# Autodesk Inventor assembly: Motor-Assembly
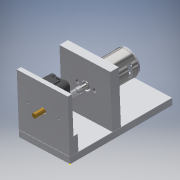
[picture p0: Inventor's stored thumbnail of the model, 180x180]
Saved by Autodesk Inventor 2016 (Build 200138000, 138)
## iProperties
Created: 2015-05-19
Part Number: Motor-Assembly
Document SubType Name: Assembly
Designer: jonathan
Author: jonathan
## Documents named in this file (3)
- C:\Users\jonathan\Desktop\CLEAN COPIES\DC Motor Test Stand\Inventor\DC Motor Test Stand.iam
- C:\Users\jonathan\Desktop\CLEAN COPIES\DC Motor Test Stand\Inventor\Fixture Assembly.iam
- C:\Users\jonathan\Desktop\CLEAN COPIES\DC Motor Test Stand\Inventor\Axle Assembly.iam
## Components (2 placed, 2 different names)
1. Fixture Assembly:1 [sub-assembly] — Mate:1, Mate:2
2. Axle Assembly:1 [sub-assembly] — Mate:1, Mate:2
## Relationships (2: Mate 2)
- Mate:1: Fixture Assembly:1 ↔ Axle Assembly:1
- Mate:2: Fixture Assembly:1 ↔ Axle Assembly:1
